# Autodesk Inventor assembly: Robot
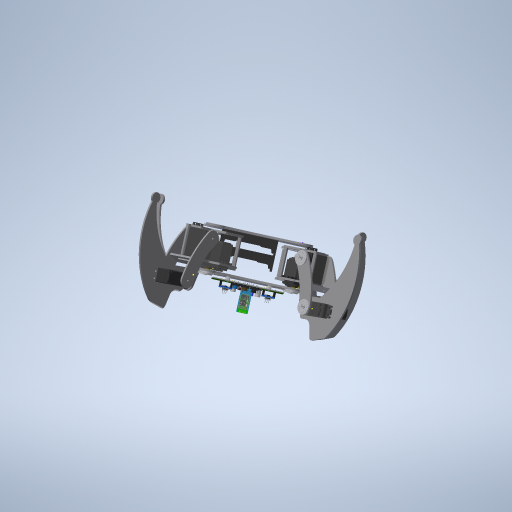
[picture p0: Inventor's stored thumbnail of the model, 512x512]
Saved by Autodesk Inventor 2024 (Build 280153000, 153)
## iProperties
Created: 2023-04-17
Part Number: Robot
Document SubType Name: Assembly
Designer: Analuam
Author: Analuam
## Documents named in this file (13)
- D:\Dek Diyah\Robot.iam
- D:\Dek Diyah\Base1.ipt
- D:\Dek Diyah\Base2.ipt
- D:\Dek Diyah\AssemblyCoxa.iam
- D:\Dek Diyah\servomg996r\Acople circular.ipt
- D:\Dek Diyah\AssemblyCoxaKa.iam
- D:\Dek Diyah\Femm.iam
- D:\Dek Diyah\Part3.ipt
- D:\Dek Diyah\Servo berputar.iam
- D:\Dek Diyah\femki.iam
- D:\Dek Diyah\Assembly9.iam
- F:\Inventor part\M3x5_Screwed_Spacer_Sleeve_(Standoff).ipt
- F:\Inventor part\BK-18650-PC4.ipt
## Components (29 placed, 12 different names)
1. Base1:1 — Mate:2, Insert:24, Mate:18
2. Base2:1 — Mate:2, Insert:1, Insert:3, Insert:5, Insert:18, Insert:19, Insert:20, Insert:21, Insert:24, Insert:25
3. AssemblyCoxa:1 [sub-assembly] — Insert:2, Insert:14
4. Acople circular:1 — Insert:1, Insert:2
5. Acople circular:2 — Insert:3, Insert:4
6. AssemblyCoxa:2 [sub-assembly] — Insert:4, Insert:15
7. AssemblyCoxaKa:1 [sub-assembly] — Insert:11, Insert:26
8. Acople circular:3 — Insert:5, Insert:8
9. Acople circular:4 — Insert:25, Insert:26
10. AssemblyCoxaKa:2 [sub-assembly] — Insert:8, Insert:9
11. Femm:1 [sub-assembly] — Insert:9, Insert:10
12. Part3:1 — Mate:4, Mate:5, Mate:6
13. Servo berputar:1 [sub-assembly] — Insert:10, Mate:4, Mate:5, Mate:6
14. Femm:2 [sub-assembly] — Insert:11, Insert:13
15. Servo berputar:2 [sub-assembly] — Insert:13, Mate:7, Mate:8, Mate:9
16. Part3:2 — Mate:7, Mate:8, Mate:9
17. femki:1 [sub-assembly] — Insert:14, Insert:17
18. femki:2 [sub-assembly] — Insert:15, Insert:16
19. Servo berputar:3 [sub-assembly] — Insert:16, Mate:10, Mate:11, Mate:12
20. Servo berputar:4 [sub-assembly] — Insert:17, Mate:13, Mate:14, Mate:15
21. Part3:3 — Mate:10, Mate:11, Mate:12
22. Part3:4 — Mate:13, Mate:14, Mate:15
23. Assembly9:1 [sub-assembly] — Insert:22, Insert:23, Flush:3
24. M3x5_Screwed_Spacer_Sleeve_(Standoff):1 — Insert:20
25. M3x5_Screwed_Spacer_Sleeve_(Standoff):2 — Insert:18
26. M3x5_Screwed_Spacer_Sleeve_(Standoff):3 — Insert:19, Insert:23
27. M3x5_Screwed_Spacer_Sleeve_(Standoff):4 — Insert:21, Insert:22
28. BK-18650-PC4:1 — Flush:1, Flush:2, Mate:17, Mate:18
29. BK-18650-PC4:2 — Flush:1, Flush:2, Mate:17, Flush:3
## Relationships (41: Insert 23, Mate 15, Flush 3)
- Mate:2: Base1:1 ↔ Base2:1
- Insert:1: Base2:1 ↔ Acople circular:1
- Insert:2: AssemblyCoxa:1 ↔ Acople circular:1
- Insert:3: Base2:1 ↔ Acople circular:2
- Insert:4: Acople circular:2 ↔ AssemblyCoxa:2
- Insert:5: Base2:1 ↔ Acople circular:3
- Insert:8: Acople circular:3 ↔ AssemblyCoxaKa:2
- Insert:9: AssemblyCoxaKa:2 ↔ Femm:1
- Insert:10: Femm:1 ↔ Servo berputar:1
- Mate:4: Part3:1 ↔ Servo berputar:1
- Mate:5: Part3:1 ↔ Servo berputar:1
- Mate:6: Part3:1 ↔ Servo berputar:1
- Insert:11: AssemblyCoxaKa:1 ↔ Femm:2
- Insert:13: Femm:2 ↔ Servo berputar:2
- Mate:7: Servo berputar:2 ↔ Part3:2
- Mate:8: Servo berputar:2 ↔ Part3:2
- Mate:9: Servo berputar:2 ↔ Part3:2
- Insert:14: AssemblyCoxa:1 ↔ femki:1
- Insert:15: AssemblyCoxa:2 ↔ femki:2
- Insert:16: femki:2 ↔ Servo berputar:3
- Insert:17: femki:1 ↔ Servo berputar:4
- Mate:10: Servo berputar:3 ↔ Part3:3
- Mate:11: Servo berputar:3 ↔ Part3:3
- Mate:12: Servo berputar:3 ↔ Part3:3
- Mate:13: Servo berputar:4 ↔ Part3:4
- Mate:14: Servo berputar:4 ↔ Part3:4
- Mate:15: Servo berputar:4 ↔ Part3:4
- Insert:18: Base2:1 ↔ M3x5_Screwed_Spacer_Sleeve_(Standoff):2
- Insert:19: Base2:1 ↔ M3x5_Screwed_Spacer_Sleeve_(Standoff):3
- Insert:20: Base2:1 ↔ M3x5_Screwed_Spacer_Sleeve_(Standoff):1
- Insert:21: Base2:1 ↔ M3x5_Screwed_Spacer_Sleeve_(Standoff):4
- Insert:22: Assembly9:1 ↔ M3x5_Screwed_Spacer_Sleeve_(Standoff):4
- Insert:23: Assembly9:1 ↔ M3x5_Screwed_Spacer_Sleeve_(Standoff):3
- Insert:24 (60 mm): Base1:1 ↔ Base2:1
- Insert:25: Base2:1 ↔ Acople circular:4
- Insert:26: AssemblyCoxaKa:1 ↔ Acople circular:4
- Flush:1: BK-18650-PC4:1 ↔ BK-18650-PC4:2
- Flush:2: BK-18650-PC4:1 ↔ BK-18650-PC4:2
- Mate:17: BK-18650-PC4:1 ↔ BK-18650-PC4:2
- Mate:18: Base1:1 ↔ BK-18650-PC4:1
- Flush:3: Assembly9:1 ↔ BK-18650-PC4:2
